# Autodesk Inventor assembly: Troysassembly1
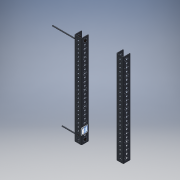
[picture p0: Inventor's stored thumbnail of the model, 180x180]
Saved by Autodesk Inventor 2016 (Build 200138000, 138)
## iProperties
Created: 2015-09-25
Part Number: Troysassembly1
Document SubType Name: Assembly
Designer: phi
Author: phi
## Documents named in this file (4)
- C:\Users\phi\Documents\GitHub\phi_robotics\3d-models\FTC_Tetrix_KOP_Block_Party\Troysassembly1.iam
- C:\Users\phi\Documents\GitHub\phi_robotics\3d-models\FTC_Tetrix_KOP_Block_Party\Tetrix_Kit_FTC\Autodesk Inventor Files\tetrix_c_channel-5.ipt
- C:\Users\phi\Documents\GitHub\phi_robotics\3d-models\FTC_Tetrix_KOP_Block_Party\Tetrix_Kit_FTC\Autodesk Inventor Files\tetrix_axle.ipt
- C:\Users\phi\Documents\GitHub\phi_robotics\3d-models\FTC_Tetrix_KOP_Block_Party\Tetrix_Kit_FTC\Autodesk Inventor Files\tetrix_bushing.ipt
## Components (8 placed, 3 different names)
1. tetrix_c_channel-5:1 — Rigid:1, Rigid:2, Rigid:3, Rigid:4
2. tetrix_c_channel-5:2
3. tetrix_bushing:8 — Rigid:1
4. tetrix_bushing:9 — Rigid:2
5. tetrix_bushing:10 — Rigid:4, Rigid:5
6. tetrix_bushing:11 — Rigid:3
7. tetrix_axle:1 — Rigid:5
8. tetrix_axle:2
## Relationships (5: WeldJoint 5)
- Rigid:1 [WeldJoint]: tetrix_c_channel-5:1 ↔ tetrix_bushing:8
- Rigid:2 [WeldJoint]: tetrix_c_channel-5:1 ↔ tetrix_bushing:9
- Rigid:3 [WeldJoint]: tetrix_c_channel-5:1 ↔ tetrix_bushing:11
- Rigid:4 [WeldJoint]: tetrix_c_channel-5:1 ↔ tetrix_bushing:10
- Rigid:5 [WeldJoint] (5 mm): tetrix_bushing:10 ↔ tetrix_axle:1
